# Autodesk Inventor assembly: controlunit
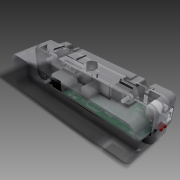
[picture p0: Inventor's stored thumbnail of the model, 180x180]
Saved by Autodesk Inventor 2014 SP1 (Build 180222100, 222)
## iProperties
Created: 2014-04-06
Part Number: controlunit
Document SubType Name: Assembly
Designer: Tyler
Author: Tyler
## Documents named in this file (5)
- C:\Users\Tyler\Documents\housing\controlunit.iam
- C:\Users\Tyler\Documents\housing\case_rear.ipt
- C:\Users\Tyler\Documents\housing\PCB\PCB.iam
- C:\Users\Tyler\Documents\housing\case_front.ipt
- C:\Users\Tyler\Documents\Inventor\Content Center Files\R2014\en-US\AS 1427(05)\AS 1427 - M3 x 8(5) II.ipt
## Components (6 placed, 4 different names)
1. case_rear:1 — Mate:1, Mate:2, Mate:3, Flush:1, Flush:2, Mate:4, Insert:1, Insert:2, Insert:3
2. PCB:1 [sub-assembly] — Mate:1, Mate:2, Mate:3
3. case_front:1 — Flush:1, Flush:2, Mate:4
4. AS 1427 H - Metric M3 x 8:1 — Insert:3
5. AS 1427 H - Metric M3 x 8:2 — Insert:2
6. AS 1427 H - Metric M3 x 8:3 — Insert:1
## Relationships (9: Mate 4, Insert 3, Flush 2)
- Mate:1: case_rear:1 ↔ PCB:1
- Mate:2: case_rear:1 ↔ PCB:1
- Mate:3: case_rear:1 ↔ PCB:1
- Flush:1: case_rear:1 ↔ case_front:1
- Flush:2: case_rear:1 ↔ case_front:1
- Mate:4: case_rear:1 ↔ case_front:1
- Insert:1: case_rear:1 ↔ AS 1427 H - Metric M3 x 8:3
- Insert:2: case_rear:1 ↔ AS 1427 H - Metric M3 x 8:2
- Insert:3: case_rear:1 ↔ AS 1427 H - Metric M3 x 8:1
